# Autodesk Inventor assembly: 前足
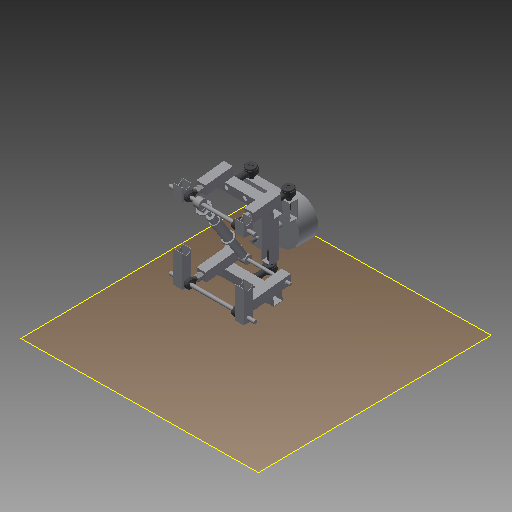
[picture p0: Inventor's stored thumbnail of the model, 512x512]
Saved by Autodesk Inventor 2018 (Build 220112000, 112)
## iProperties
Created: 2017-09-13
Part Number: 前足
Material: 一般
Document SubType Name: Assembly
Designer: mura5
Author: mura5
## Documents named in this file (14)
- D:\Works\RBBR\cart\前足改\後足.iam
- D:\Works\RBBR\cart\前足改\Aアーム下.iam
- D:\Works\RBBR\cart\iko_POS_12\AIS2014\POS 12.iam
- D:\Works\RBBR\cart\前足改\軸.ipt
- D:\Works\RBBR\cart\スプリング\スプリング.iam
- D:\Works\RBBR\cart\前足改\軸10mm.ipt
- D:\Works\RBBR\cart\iko_LHSA_14\AIS2016\LHSA 14.iam
- D:\Works\RBBR\cart\前足改\前輪ハブ.ipt
- C:\Users\mura5\Documents\RBBR\cart\前足改\車軸受け改\車軸受け.iam
- D:\Works\RBBR\cart\前足改\軸受上用.ipt
- D:\Works\RBBR\cart\前足改\軸受下用.ipt
- D:\Works\RBBR\cart\前足改\前輪シャフト.ipt
- D:\Works\RBBR\cart\前足改\Aアーム上_後.iam
- D:\Works\RBBR\cart\前足改\車軸受け改改\車軸受け_後.iam
## Components (21 placed, 13 different names)
1. Aアーム上_後:1 [sub-assembly] — 回転:1, 回転:2, リジッド:18, 回転:18, 角度:10
2. Aアーム下:2 [sub-assembly] — 回転:3, 回転:4, 角度:1, 角度:2, リジッド:2, 円柱状:8, フラッシュ:3
3. POS 12:1 [sub-assembly] — 回転:1, 円柱状:1, メイト:9, メイト:10
4. POS 12:2 [sub-assembly] — 回転:2, 円柱状:2, メイト:11
5. POS 12:3 [sub-assembly] — 回転:3, 円柱状:4, メイト:12
6. POS 12:4 [sub-assembly] — 回転:4, 円柱状:3, メイト:13
7. 軸:1 — 円柱状:1, 円柱状:2, メイト:1, フラッシュ:2, 円柱状:6, メイト:4, 円柱状:10, 円柱状:12, フラッシュ:5
8. 前輪ハブ:1 — 角度:4, 回転:15, 回転:16
9. 軸:2 — メイト:1, フラッシュ:2, メイト:2, 円柱状:3, 円柱状:4, メイト:5, メイト:6, 円柱状:11, 円柱状:13, フラッシュ:4
10. スプリング:1 [sub-assembly] — 円柱状:6, 円柱状:7, メイト:9
11. 軸10mm:1 — 円柱状:7, 円柱状:8, フラッシュ:3
12. LHSA 14:2 [sub-assembly] — リジッド:2, リジッド:11, 円柱状:14, メイト:14
13. 車軸受け:3 [sub-assembly] — リジッド:11
14. 軸受上用:1 — 円柱状:10, 角度:6, メイト:11, フラッシュ:5
15. 軸受下用:1 — 円柱状:11, 角度:7, メイト:13
16. 軸受上用:2 — 円柱状:12, メイト:10, 角度:8
17. 軸受下用:2 — 円柱状:13, メイト:12, 角度:9, フラッシュ:4
18. 車軸受け_後:1 [sub-assembly] — 回転:15, 回転:20, 回転:21, 回転:22, 円柱状:14, メイト:14
19. 前輪シャフト:1 — 回転:16
20. LHSA 14:3 [sub-assembly] — リジッド:18, 回転:21
21. LHSA 14:4 [sub-assembly] — 回転:18, 回転:20, 回転:22, 角度:10
## Relationships (49: CylindricalJoint 12, Mate 11, RevoluteJoint 10, Angle 9, Flush 4, WeldJoint 3)
- 回転:1 [RevoluteJoint] (10 mm): Aアーム上_後:1 ↔ POS 12:1
- 回転:2 [RevoluteJoint] (10 mm): Aアーム上_後:1 ↔ POS 12:2
- 回転:3 [RevoluteJoint] (10 mm): Aアーム下:2 ↔ POS 12:3
- 回転:4 [RevoluteJoint] (10 mm): Aアーム下:2 ↔ POS 12:4
- 円柱状:1 [CylindricalJoint]: POS 12:1 ↔ 軸:1
- 円柱状:2 [CylindricalJoint]: POS 12:2 ↔ 軸:1
- メイト:1 [Mate] (265 mm): 軸:1 ↔ 軸:2
- フラッシュ:2 [Flush]: 軸:1 ↔ 軸:2
- メイト:2 [Mate]: 軸:2
- 円柱状:3 [CylindricalJoint]: POS 12:4 ↔ 軸:2
- 円柱状:4 [CylindricalJoint]: POS 12:3 ↔ 軸:2
- 角度:1 [Angle] (180 deg): Aアーム下:2
- 角度:2 [Angle] (18 deg): Aアーム下:2
- 円柱状:6 [CylindricalJoint]: 軸:1 ↔ スプリング:1
- 円柱状:7 [CylindricalJoint]: スプリング:1 ↔ 軸10mm:1
- メイト:4 [Mate]: 軸:1
- メイト:5 [Mate]: 軸:2
- メイト:6 [Mate]: 軸:2
- リジッド:2 [WeldJoint]: Aアーム下:2 ↔ LHSA 14:2
- 円柱状:8 [CylindricalJoint]: Aアーム下:2 ↔ 軸10mm:1
- リジッド:11 [WeldJoint]: LHSA 14:2 ↔ 車軸受け:3
- メイト:9 [Mate] (20 mm): POS 12:1 ↔ スプリング:1
- 角度:4 [Angle] (180 deg): 前輪ハブ:1
- 角度:5 [Angle] (0 deg)
- 円柱状:10 [CylindricalJoint]: 軸:1 ↔ 軸受上用:1
- 角度:6 [Angle] (180 deg): 軸受上用:1
- 円柱状:11 [CylindricalJoint]: 軸:2 ↔ 軸受下用:1
- 角度:7 [Angle] (180 deg): 軸受下用:1
- 円柱状:12 [CylindricalJoint]: 軸:1 ↔ 軸受上用:2
- メイト:10 [Mate]: POS 12:1 ↔ 軸受上用:2
- メイト:11 [Mate]: POS 12:2 ↔ 軸受上用:1
- 角度:8 [Angle] (180 deg): 軸受上用:2
- 円柱状:13 [CylindricalJoint]: 軸:2 ↔ 軸受下用:2
- メイト:12 [Mate]: POS 12:3 ↔ 軸受下用:2
- メイト:13 [Mate]: POS 12:4 ↔ 軸受下用:1
- 角度:9 [Angle] (180 deg): 軸受下用:2
- フラッシュ:3 [Flush] (15 mm): Aアーム下:2 ↔ 軸10mm:1
- フラッシュ:4 [Flush] (26 mm): 軸:2 ↔ 軸受下用:2
- フラッシュ:5 [Flush] (26 mm): 軸:1 ↔ 軸受上用:1
- 回転:15 [RevoluteJoint]: 前輪ハブ:1 ↔ 車軸受け_後:1
- 回転:16 [RevoluteJoint]: 前輪ハブ:1 ↔ 前輪シャフト:1
- リジッド:18 [WeldJoint]: Aアーム上_後:1 ↔ LHSA 14:3
- 回転:18 [RevoluteJoint]: Aアーム上_後:1 ↔ LHSA 14:4
- 回転:20 [RevoluteJoint]: 車軸受け_後:1 ↔ LHSA 14:4
- 回転:21 [RevoluteJoint]: 車軸受け_後:1 ↔ LHSA 14:3
- 回転:22 [RevoluteJoint]: 車軸受け_後:1 ↔ LHSA 14:4
- 角度:10 [Angle] (0 deg): Aアーム上_後:1 ↔ LHSA 14:4
- 円柱状:14 [CylindricalJoint]: LHSA 14:2 ↔ 車軸受け_後:1
- メイト:14 [Mate]: LHSA 14:2 ↔ 車軸受け_後:1
